# Autodesk Inventor assembly: Extruder Assembky
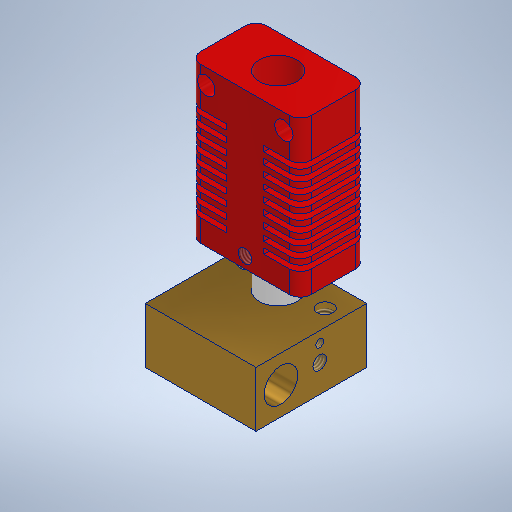
[picture p0: Inventor's stored thumbnail of the model, 512x512]
Saved by Autodesk Inventor 2025 (Build 290162000, 162)
## iProperties
Created: 2025-03-12
Part Number: Extruder Assembky
Document SubType Name: Assembly
Designer: MAL16204
Author: MAL16204
## Documents named in this file (3)
- C:\Users\MAL16204\OneDrive - Pennsylvania Western University\Spring 2025\MECH 2400\CAD Projects\Final Project\Extruder Assembky.iam
- C:\Users\MAL16204\OneDrive - Pennsylvania Western University\Spring 2025\MECH 2400\CAD Projects\Final Project\Hotend.ipt
- C:\Users\MAL16204\OneDrive - Pennsylvania Western University\Spring 2025\MECH 2400\CAD Projects\Final Project\Nozzle 0.4mm.ipt
## Components (2 placed, 2 different names)
1. Hotend:1 — Cylindrical:1
2. Nozzle 0.4mm:1 — Cylindrical:1
## Relationships (1: CylindricalJoint 1)
- Cylindrical:1: Hotend:1 ↔ Nozzle 0.4mm:1
